# Autodesk Inventor assembly: Body
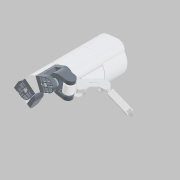
[picture p0: Inventor's stored thumbnail of the model, 180x180]
Saved by Autodesk Inventor 2017 (Build 210142000, 142)
## iProperties
Created: 2017-03-13
Part Number: Body
Document SubType Name: Assembly
Designer: zallen
Author: zallen
## Documents named in this file (5)
- C:\Users\zallen\Documents\GitHub\cr-laundry-robot\src\Body\Body.iam
- C:\Users\zallen\Documents\GitHub\cr-laundry-robot\src\Body\Arm Assembly\ArmAssembly.iam
- C:\Users\zallen\Documents\GitHub\cr-laundry-robot\src\Body\Chest Assembly\Chest Assembly.iam
- C:\Users\zallen\Documents\GitHub\cr-laundry-robot\src\Body\Bucket Assembly\Bucket Assembly.iam
- C:\Users\zallen\Documents\GitHub\cr-laundry-robot\src\Body\Spine Assembly\Spine Assembly.iam
## Components (5 placed, 4 different names)
1. ArmAssembly:1 [sub-assembly] — Mate:16, Mate:34, Mate:35
2. ArmAssembly:2 [sub-assembly] — Mate:17, Mate:19, Mate:30, Mate:32
3. Chest Assembly:1 [sub-assembly] — Mate:16, Mate:17, Mate:19, Mate:24, Mate:25, Mate:26, Mate:27, Mate:32, Mate:34, Mate:35
4. Bucket Assembly:1 [sub-assembly] — Mate:11, Mate:12, Mate:13, Mate:14, Mate:23, Mate:28, Mate:29
5. Spine Assembly:1 [sub-assembly] — Mate:23, Mate:24, Mate:25, Mate:26, Mate:27, Mate:28, Mate:29
## Relationships (18: Mate 18)
- Mate:11: Bucket Assembly:1
- Mate:12: Bucket Assembly:1
- Mate:13: Bucket Assembly:1
- Mate:14: Bucket Assembly:1
- Mate:16: ArmAssembly:1 ↔ Chest Assembly:1
- Mate:17: ArmAssembly:2 ↔ Chest Assembly:1
- Mate:19: ArmAssembly:2 ↔ Chest Assembly:1
- Mate:23: Bucket Assembly:1 ↔ Spine Assembly:1
- Mate:24: Chest Assembly:1 ↔ Spine Assembly:1
- Mate:25: Chest Assembly:1 ↔ Spine Assembly:1
- Mate:26: Chest Assembly:1 ↔ Spine Assembly:1
- Mate:27: Chest Assembly:1 ↔ Spine Assembly:1
- Mate:28: Bucket Assembly:1 ↔ Spine Assembly:1
- Mate:29: Bucket Assembly:1 ↔ Spine Assembly:1
- Mate:30: ArmAssembly:2
- Mate:32: ArmAssembly:2 ↔ Chest Assembly:1
- Mate:34: ArmAssembly:1 ↔ Chest Assembly:1
- Mate:35: ArmAssembly:1 ↔ Chest Assembly:1
